# Autodesk Inventor assembly: HipRightNCS
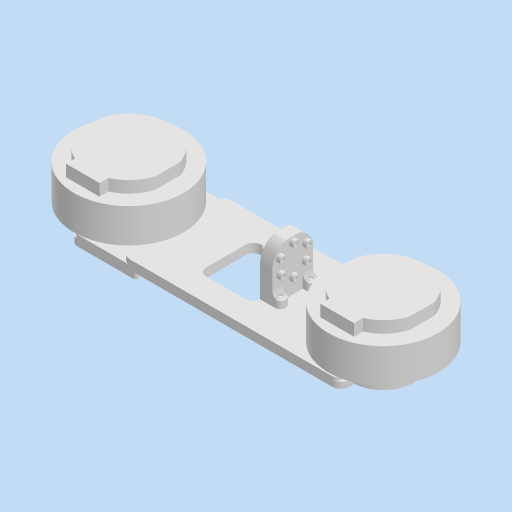
[picture p0: Inventor's stored thumbnail of the model, 512x512]
Saved by Autodesk Inventor 2023 (Build 270158000, 158)
## iProperties
Created: 2026-06-18
Part Number: HipRightNCS
Document SubType Name: Assembly
Designer: Nathann
Author: Nathann
## Documents named in this file (2)
- C:\Users\Nathann\ClawdDrive\Objet3D\RunningRobot\PartURDF\HipRightNCS.iam
- C:\Users\Nathann\ClawdDrive\Objet3D\RunningRobot\PartURDF\HipRight_Simplify_1.ipt
## Components (1 placed, 1 different names)
1. HipRight_Simplify_1:1 — Mate:1, Flush:1, Mate:2, Angle:1
## Relationships (6: Mate 4, Flush 1, Angle 1)
- Mate:1: HipRight_Simplify_1:1
- Flush:1: HipRight_Simplify_1:1
- Mate:2: HipRight_Simplify_1:1
- Mate:3
- Mate:4
- Angle:1 (180 deg): HipRight_Simplify_1:1
